# Autodesk Inventor assembly: HS 48T Gear, No Insert_CPY
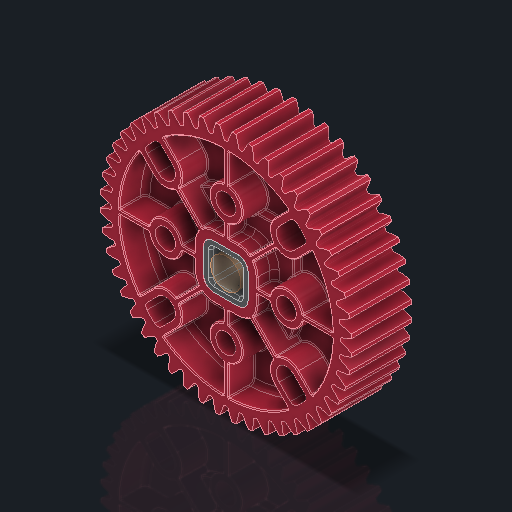
[picture p0: Inventor's stored thumbnail of the model, 512x512]
Saved by Autodesk Inventor 2023.2 (Build 272271030, 271C)
## iProperties
Created: 2022-08-02
Part Number: HS 48T Gear, No Insert_CPY
Document SubType Name: Assembly
Designer: Michael
Author: ylu12
## Documents named in this file (2)
- C:\Users\black\OneDrive\Pictures\Documents\VEX CAD\VEX-CAD-Inventor-1.4.0\Motion\Gears\HS Gear\HS 48T Gear, No Insert_CPY.iam
- C:\Users\black\OneDrive\Pictures\Documents\VEX CAD\VEX-CAD-Inventor-1.4.0\Motion\Gears\Reference Files\HS 48T Gear, No Insert_CPY.ipt
## Components (1 placed, 1 different names)
1. HS 48T Gear, No Insert_CPY:1 — Mate:12, Mate:11, Flush:6
## Relationships (3: Mate 2, Flush 1)
- Mate:12: HS 48T Gear, No Insert_CPY:1
- Mate:11: HS 48T Gear, No Insert_CPY:1
- Flush:6: HS 48T Gear, No Insert_CPY:1
